# Autodesk Inventor assembly: FemaleHeaderPin_1x6_90
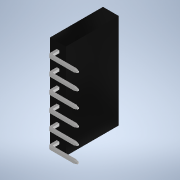
[picture p0: Inventor's stored thumbnail of the model, 180x180]
Saved by Autodesk Inventor 2021 (Build 250183000, 183)
## iProperties
Created: 2021-09-29
Part Number: FemaleHeaderPin_1x6_90
Document SubType Name: Assembly
Designer: ermoz
Author: ermoz
## Documents named in this file (2)
- D:\Moje Wyczyny\My_Poor_Projects\Sneak100_MiniSumo\minisumo-sneak100\mechanics\ElectricElements\FemaleHeaderPin_1x6_90.iam
- D:\Moje Wyczyny\My_Poor_Projects\Sneak100_MiniSumo\minisumo-sneak100\mechanics\ElectricElements\FemaleHederPin_90.ipt
## Components (6 placed, 1 different names)
1. FemaleHederPin_90:1 — Flush:1, Flush:6, Mate:1
2. FemaleHederPin_90:2 — Flush:1, Flush:2, Flush:6, Flush:7, Mate:1, Mate:2
3. FemaleHederPin_90:3 — Flush:2, Flush:3, Flush:7, Flush:8, Mate:2, Mate:3
4. FemaleHederPin_90:4 — Flush:3, Flush:4, Flush:8, Flush:9, Mate:3, Mate:4
5. FemaleHederPin_90:5 — Flush:4, Flush:5, Flush:9, Flush:10, Mate:4, Mate:5
6. FemaleHederPin_90:6 — Flush:5, Flush:10, Mate:5
## Relationships (15: Flush 10, Mate 5)
- Flush:1: FemaleHederPin_90:1 ↔ FemaleHederPin_90:2
- Flush:2: FemaleHederPin_90:2 ↔ FemaleHederPin_90:3
- Flush:3: FemaleHederPin_90:3 ↔ FemaleHederPin_90:4
- Flush:4: FemaleHederPin_90:4 ↔ FemaleHederPin_90:5
- Flush:5: FemaleHederPin_90:5 ↔ FemaleHederPin_90:6
- Flush:6: FemaleHederPin_90:1 ↔ FemaleHederPin_90:2
- Flush:7: FemaleHederPin_90:2 ↔ FemaleHederPin_90:3
- Flush:8: FemaleHederPin_90:3 ↔ FemaleHederPin_90:4
- Flush:9: FemaleHederPin_90:4 ↔ FemaleHederPin_90:5
- Flush:10: FemaleHederPin_90:5 ↔ FemaleHederPin_90:6
- Mate:1: FemaleHederPin_90:1 ↔ FemaleHederPin_90:2
- Mate:2: FemaleHederPin_90:2 ↔ FemaleHederPin_90:3
- Mate:3: FemaleHederPin_90:3 ↔ FemaleHederPin_90:4
- Mate:4: FemaleHederPin_90:4 ↔ FemaleHederPin_90:5
- Mate:5: FemaleHederPin_90:5 ↔ FemaleHederPin_90:6
